# Autodesk Inventor assembly: ASM_SensorHead_LowerSensor
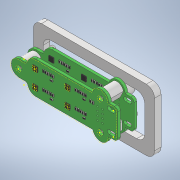
[picture p0: Inventor's stored thumbnail of the model, 180x180]
Saved by Autodesk Inventor 2022.2 (Build 262287010, 287A)
## iProperties
Created: 2024-09-30
Part Number: ASM_SensorHead_LowerSensor
Document SubType Name: Assembly
Designer: ppovolni
Author: ppovolni
## Documents named in this file (3)
- D:\3_Local_Projekte\_PaperGitHub\MiniBumblebee_LowFieldMapping\2_Calibration\21_Hardware\213_CalibrationSolenoid_CAD\Slider\Hallsensor_Mounting\ASM_SensorHead_UpperSensor.iam
- D:\3_Local_Projekte\_PaperGitHub\MiniBumblebee_LowFieldMapping\2_Calibration\21_Hardware\213_CalibrationSolenoid_CAD\Slider\Hallsensor_Mounting\SensorHead_PCBs.ipt
- D:\3_Local_Projekte\_PaperGitHub\MiniBumblebee_LowFieldMapping\2_Calibration\21_Hardware\213_CalibrationSolenoid_CAD\Slider\Hallsensor_Mounting\Holder_Cal_UpperSensor.ipt
## Components (2 placed, 2 different names)
1. Holder_Cal_UpperSensor:1 — Passend:1, Winkel:1, Winkel:2, Passend:2
2. SensorHead_PCBs:1 — Passend:1, Winkel:1, Winkel:2, Passend:2
## Relationships (4: Mate 2, Angle 2)
- Passend:1 [Mate]: Holder_Cal_UpperSensor:1 ↔ SensorHead_PCBs:1
- Winkel:1 [Angle] (0 deg): Holder_Cal_UpperSensor:1 ↔ SensorHead_PCBs:1
- Winkel:2 [Angle] (0 deg): Holder_Cal_UpperSensor:1 ↔ SensorHead_PCBs:1
- Passend:2 [Mate]: Holder_Cal_UpperSensor:1 ↔ SensorHead_PCBs:1
